# Autodesk Inventor assembly: Assembly_AIM
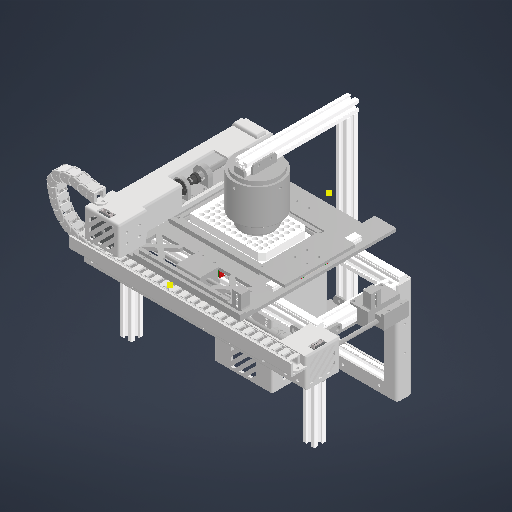
[picture p0: Inventor's stored thumbnail of the model, 512x512]
Saved by Autodesk Inventor 2026.2 (Build 302298000, 298)
## iProperties
Created: 2026-02-12
Part Number: Assembly_AIM
Document SubType Name: Assembly
Designer: Alvin
Author: Alvin
## Documents named in this file (54)
- C:\Users\Alvin\OneDrive\Documents\Inventor\NCKU_Automation_Incubator_Microscope\Assembly_AIM.iam
- C:\Users\Alvin\OneDrive\Documents\Inventor\NCKU_Automation_Incubator_Microscope\alpro base 200mm.ipt
- C:\Users\Alvin\OneDrive\Documents\Inventor\NCKU_Automation_Incubator_Microscope\alpro base 330mm.ipt
- C:\Users\Alvin\OneDrive\Documents\Inventor\NCKU_Automation_Incubator_Microscope\MGN12H_With_Rail x axis\MGN12H_With_Rail x axis.iam
- C:\Users\Alvin\OneDrive\Documents\Inventor\NCKU_Automation_Incubator_Microscope\stagex v7 new version\stagex v7 new version.iam
- C:\Users\Alvin\OneDrive\Documents\Inventor\NCKU_Automation_Incubator_Microscope\alpro base 120mm.ipt
- C:\Users\Alvin\OneDrive\Documents\Inventor\NCKU_Automation_Incubator_Microscope\bracketx.ipt
- C:\Users\Alvin\OneDrive\Documents\Inventor\NCKU_Automation_Incubator_Microscope\NEMA17 42-40\NEMA17 42-40\NEMA17 42-40.ipt
- C:\Users\Alvin\OneDrive\Documents\Inventor\NCKU_Automation_Incubator_Microscope\KFL08-KFL08-Part\KFL08-KFL08-Part.iam
- C:\Users\Alvin\OneDrive\Documents\Inventor\NCKU_Automation_Incubator_Microscope\MGN12H_With_Rail y axis\MGN12H_With_Rail y axis.iam
- C:\Users\Alvin\OneDrive\Documents\Inventor\NCKU_Automation_Incubator_Microscope\NEMA17_Coupler v1.ipt
- C:\Users\Alvin\OneDrive\Documents\Inventor\NCKU_Automation_Incubator_Microscope\8mm Threaded Rod 350mm.ipt
- C:\Users\Alvin\OneDrive\Documents\Inventor\NCKU_Automation_Incubator_Microscope\bracketx part2.ipt
- C:\Users\Alvin\OneDrive\Documents\Inventor\NCKU_Automation_Incubator_Microscope\anti-baclash nuts v1\anti-baclash nuts v1.iam
- C:\Users\Alvin\OneDrive\Documents\Inventor\NCKU_Automation_Incubator_Microscope\microswith.ipt
- C:\Users\Alvin\OneDrive\Documents\Inventor\NCKU_Automation_Incubator_Microscope\limitswitch_bracket_2 v1.ipt
- C:\Users\Alvin\OneDrive\Documents\Inventor\NCKU_Automation_Incubator_Microscope\plate assembly\plate assembly.iam
- C:\Users\Alvin\OneDrive\Documents\Inventor\NCKU_Automation_Incubator_Microscope\kfl_bracket_2 v1.ipt
- C:\Users\Alvin\OneDrive\Documents\Inventor\NCKU_Automation_Incubator_Microscope\brackety.ipt
- C:\Users\Alvin\OneDrive\Documents\Inventor\NCKU_Automation_Incubator_Microscope\8mm Threaded Rod 170mm.ipt
- C:\Users\Alvin\OneDrive\Documents\Inventor\NCKU_Automation_Incubator_Microscope\alpro base 290mm.ipt
- C:\Users\Alvin\OneDrive\Documents\Inventor\NCKU_Automation_Incubator_Microscope\z part new version.ipt
- C:\Users\Alvin\OneDrive\Documents\Inventor\NCKU_Automation_Incubator_Microscope\kfl_bracket v3.ipt
- C:\Users\Alvin\OneDrive\Documents\Inventor\NCKU_Automation_Incubator_Microscope\well plate\96 Well Plate, F-bottom, Standard v2.ipt
- C:\Users\Alvin\OneDrive\Documents\Inventor\NCKU_Automation_Incubator_Microscope\alpro base 400mm v4.ipt
- C:\Users\Alvin\OneDrive\Documents\Inventor\NCKU_Automation_Incubator_Microscope\8mm Threaded Rod 101.5mm.ipt
- C:\Users\Alvin\OneDrive\Documents\Inventor\NCKU_Automation_Incubator_Microscope\Metal rod 108mm (6mm).ipt
- C:\Users\Alvin\OneDrive\Documents\Inventor\NCKU_Automation_Incubator_Microscope\LMF8_fix.ipt
- C:\Users\Alvin\OneDrive\Documents\Inventor\NCKU_Automation_Incubator_Microscope\IModule_Mounting Part-2.ipt
- C:\Users\Alvin\OneDrive\Documents\Inventor\NCKU_Automation_Incubator_Microscope\IModule_Mounting Part-3.ipt
- C:\Users\Alvin\OneDrive\Documents\Inventor\NCKU_Automation_Incubator_Microscope\IModule_LED.ipt
- C:\Users\Alvin\OneDrive\Documents\Inventor\NCKU_Automation_Incubator_Microscope\IModule_Diffuser.ipt
- C:\Users\Alvin\OneDrive\Documents\Inventor\NCKU_Automation_Incubator_Microscope\IModule_CollectorLens.ipt
- C:\Users\Alvin\OneDrive\Documents\Inventor\NCKU_Automation_Incubator_Microscope\alpro base 220mm v4.ipt
- C:\Users\Alvin\OneDrive\Documents\Inventor\NCKU_Automation_Incubator_Microscope\IModule_Mounting Part-1.ipt
- C:\Users\Alvin\OneDrive\Documents\Inventor\NCKU_Automation_Incubator_Microscope\metal rod 180mm.ipt
- C:\Users\Alvin\OneDrive\Documents\Inventor\NCKU_Automation_Incubator_Microscope\10x Obj Lens Finite 160mm.ipt
- C:\Users\Alvin\OneDrive\Documents\Inventor\NCKU_Automation_Incubator_Microscope\z part 2 new version_1.ipt
- C:\Users\Alvin\OneDrive\Documents\Inventor\NCKU_Automation_Incubator_Microscope\Tube_ObjLens+RaspiCam.iam
- C:\Users\Alvin\OneDrive\Documents\Inventor\NCKU_Automation_Incubator_Microscope\raspberry-pi-global-shutter-camera-1.snapshot.4\Raspberry Pi Global Shutter Camera\Raspberry Pi Global Shutter Camera\Raspberry Pi.ipt
- C:\Users\Alvin\OneDrive\Documents\Inventor\NCKU_Automation_Incubator_Microscope\z_enclosure.ipt
- C:\Users\Alvin\OneDrive\Documents\Inventor\NCKU_Automation_Incubator_Microscope\xy_enclosure.ipt
- C:\Users\Alvin\OneDrive\Documents\Inventor\NCKU_Automation_Incubator_Microscope\x_enclosure.ipt
- C:\Users\Alvin\OneDrive\Documents\Inventor\NCKU_Automation_Incubator_Microscope\enclosure__bone_bottom.ipt
- C:\Users\Alvin\OneDrive\Documents\Inventor\NCKU_Automation_Incubator_Microscope\enclosure__bone_bottom_left.ipt
- C:\Users\Alvin\OneDrive\Documents\Inventor\NCKU_Automation_Incubator_Microscope\metal rod 80mm.ipt
- C:\Users\Alvin\OneDrive\Documents\Inventor\NCKU_Automation_Incubator_Microscope\chain_cable_male.ipt
- C:\Users\Alvin\OneDrive\Documents\Inventor\NCKU_Automation_Incubator_Microscope\chain_cable_mid.ipt
- C:\Users\Alvin\OneDrive\Documents\Inventor\NCKU_Automation_Incubator_Microscope\chain_cable_female.ipt
- C:\Users\Alvin\OneDrive\Documents\Inventor\NCKU_Automation_Incubator_Microscope\Assembly_AIM\AIP\FEA\feo31tnmo.fins
- C:\Users\Alvin\OneDrive\Documents\Inventor\NCKU_Automation_Incubator_Microscope\Assembly_AIM\AIP\FEA\feo31tnmo.fsat
- C:\Users\Alvin\OneDrive\Documents\Inventor\NCKU_Automation_Incubator_Microscope\Assembly_AIM\AIP\FEA\feo31tnmo.ftes
- C:\Users\Alvin\OneDrive\Documents\Inventor\NCKU_Automation_Incubator_Microscope\Assembly_AIM\AIP\FEA\feo31tnmo.fwiz
- C:\Users\Alvin\OneDrive\Documents\Inventor\NCKU_Automation_Incubator_Microscope\Assembly_AIM\AIP\FEA\feo31tq5c.fmsh
## Components (97 placed, 48 different names)
1. alpro base 330mm:1 — Flush:15, Flush:17, Mate:10, Mate:13, Flush:19, Flush:20, Mate:15, Flush:23, Flush:24, Mate:21, Flush:27, Mate:94, Flush:37, Mate:200, Flush:45, Flush:46, Mate:201, Flush:47, Flush:48
2. alpro base 330mm:2 — Flush:16, Flush:18, Mate:11, Mate:14, Flush:21, Flush:22, Mate:16, Flush:25, Flush:26, Mate:198, Flush:41, Flush:42, Mate:199, Flush:43, Flush:44
3. MGN12H_With_Rail x axis:1 [sub-assembly] — Flush:16, Flush:18, Mate:11, Mate:302, Mate:303, Mate:304
4. MGN12H_With_Rail x axis:2 [sub-assembly] — Flush:15, Flush:17, Mate:10, Mate:84
5. alpro base 120mm:1 — Mate:13, Flush:19, Flush:20, Mate:16, Flush:25, Flush:26, Mate:93
6. alpro base 120mm:2 — Mate:14, Flush:21, Flush:22, Mate:15, Flush:23, Flush:24, Mate:20, Mate:328, Mate:329
7. bracketx:1 — Mate:20, Mate:21, Flush:27, Mate:23, Mate:24, Mate:171, Mate:321, Mate:333
8. NEMA17 42-40:1 — Mate:23, Mate:24, Mate:38, Flush:29, Mate:171, Mate:335
9. NEMA17 42-40:2 — Mate:83, Flush:36, Mate:103, Mate:104, Mate:105, Mate:106, Mate:107
10. NEMA17 42-40:3 — Flush:30, Mate:56, Mate:284, Mate:285, Mate:286
11. MGN12H_With_Rail y axis:1 [sub-assembly] — Mate:58, Mate:59, Mate:290, Mate:291, Mate:292
12. MGN12H_With_Rail y axis:2 [sub-assembly] — Mate:57, Mate:60, Mate:61, Mate:287, Mate:288, Mate:289
13. NEMA17_Coupler v1:1 — Mate:83, Flush:36, Mate:118, Mate:119, Rotation:3, Mate:277
14. NEMA17_Coupler v1:2 — Flush:30, Mate:56, Cylindrical:5, Mate:75, Rotation:2
15. NEMA17_Coupler v1:3 — Mate:38, Flush:29, Cylindrical:2, Mate:39, Rotation:1
16. 8mm Threaded Rod 350mm:1 — Cylindrical:2, Mate:39, Rotation:1, Mate:45, Rotation/Translation:1, Mate:279
17. bracketx part2:1 — Mate:40, Mate:41, Mate:42, Mate:43, Mate:44, Rotation/Translation:1, Mate:84, Mate:195, Mate:196, Mate:296, Mate:297, Mate:298
18. anti-baclash nuts v1:1 [sub-assembly] — Mate:40, Mate:41, Mate:42, Mate:43, Mate:44, Mate:45
19. anti-baclash nuts v1:2 [sub-assembly] — Cylindrical:3, Mate:421, Mate:422, Mate:423
20. microswith:1 — Mate:299, Mate:301, Mate:316
21. microswith:2 — Mate:330, Mate:331, Mate:332
22. plate assembly:1 [sub-assembly] — Mate:57, Mate:58, Mate:59, Mate:60, Mate:61, Mate:233, Mate:234, Mate:235, Mate:418, Mate:419, Mate:420
23. kfl_bracket_2 v1:1 — Mate:71, Mate:72, Mate:73, Mate:74, Mate:305, Mate:306, Mate:309, Mate:416
24. KFL08-KFL08-Part:2 [sub-assembly] — Mate:71, Mate:72, Mate:73, Mate:74, Cylindrical:4
25. 8mm Threaded Rod 170mm:1 — Cylindrical:3, Cylindrical:4, Cylindrical:5, Mate:75, Rotation:2
26. kfl_bracket v3:1 — Mate:93, Mate:94, Flush:37, Mate:280, Mate:281, Mate:282
27. 96 Well Plate, F-bottom, Standard v2:1 — Mate:233, Mate:234, Mate:235
28. z part new version:1 — Mate:103, Mate:104, Mate:105, Mate:106, Mate:107, Mate:108, Flush:38, Mate:109, Mate:111, Mate:112, Mate:113, Mate:114, Mate:115, Mate:116, Mate:117, Mate:255, Mate:256, Flush:51, Flush:52, Mate:276, Mate:326, Mate:429
29. alpro base 400mm v4:1 — Mate:108, Flush:38, Mate:109, Mate:143, Flush:39, Flush:40
30. 8mm Threaded Rod 101.5mm:1 — Mate:117, Mate:118, Mate:119, Mate:140, Rotation:3
31. Metal rod 108mm (6mm):1 — Mate:111, Mate:112, Mate:113, Mate:142
32. Metal rod 108mm (6mm):2 — Mate:114, Mate:115, Mate:116, Mate:141
33. LMF8_fix:1 — Mate:142, Mate:262, Mate:267, Mate:268
34. LMF8_fix:2 — Mate:141, Mate:263, Mate:265, Mate:270
35. anti-baclash nuts v1:3 [sub-assembly] — Mate:140, Mate:264, Mate:266, Mate:269
36. alpro base 220mm v4:1 — Mate:143, Flush:39, Flush:40, Mate:163, Mate:244
37. IModule_CollectorLens:1 — Mate:149, Mate:153, Mate:154, Mate:155, Mate:156
38. IModule_Diffuser:1 — Mate:144, Mate:145
39. IModule_LED:1 — Mate:146, Mate:147, Mate:186, Mate:187
40. IModule_Mounting Part-1:1 — Mate:146, Mate:147, Mate:149, Mate:153, Mate:154, Mate:155, Mate:156, Mate:157, Mate:158, Mate:159, Mate:160, Mate:163, Mate:186, Mate:187, Mate:244
41. IModule_Mounting Part-2:1 — Mate:144, Mate:145, Mate:157, Mate:158, Mate:159, Mate:160, Mate:240, Mate:241, Mate:242, Mate:243, Mate:275, Mate:317
42. metal rod 180mm:1 — Mate:195, Mate:196, Mate:293, Mate:294, Mate:295
43. alpro base 200mm:1 — Mate:198, Flush:41, Flush:42, Flush:54, Mate:326
44. alpro base 200mm:2 — Mate:200, Flush:45, Flush:46
45. alpro base 200mm:3 — Mate:199, Flush:43, Flush:44, Mate:254, Flush:49, Flush:50, Mate:324
46. alpro base 200mm:4 — Mate:201, Flush:47, Flush:48
47. Raspberry Pi:1 — Mate:259, Mate:260, Mate:272, Mate:273, Mate:274
48. IModule_Mounting Part-3:1 — Mate:240, Mate:241, Mate:242, Mate:243
49. alpro base 290mm:1 — Mate:254, Flush:49, Flush:50, Mate:255, Mate:256, Mate:323, Flush:55, Mate:325
50. 10x Obj Lens Finite 160mm:1 — Mate:257, Mate:258, Mate:275, Mate:317
51. Tube_ObjLens+RaspiCam:1 [sub-assembly] — Mate:257, Mate:258, Mate:259, Mate:260, Mate:271
52. z part 2 new version_1:1 — Mate:262, Mate:263, Mate:264, Mate:265, Mate:266, Mate:267, Mate:268, Mate:269, Mate:270, Mate:271, Mate:272, Mate:273, Mate:274, Mate:277
53. z_enclosure:1 — Flush:51, Flush:52, Mate:276
54. KFL08-KFL08-Part:3 [sub-assembly] — Mate:279, Mate:280, Mate:281, Mate:282
55. stagex v7 new version:1 [sub-assembly] — Mate:284, Mate:285, Mate:286, Mate:287, Mate:288, Mate:289, Mate:290, Mate:291, Mate:292, Mate:293, Mate:294, Mate:295, Mate:296, Mate:297, Mate:298, Mate:299, Mate:301, Mate:302, Mate:303, Mate:304, Mate:305, Mate:306, Mate:309, Mate:316, Mate:416, Mate:424, Mate:425, Mate:426
56. x_enclosure:1 — Mate:321, Mate:370, Mate:371, Mate:415
57. enclosure__bone_bottom:1 — Flush:54, Mate:323
58. enclosure__bone_bottom_left:1 — Flush:55, Mate:324, Mate:325, Mate:429
59. limitswitch_bracket_2 v1:1 — Mate:328, Mate:329, Mate:330, Mate:331, Mate:332, Flush:56
60. metal rod 80mm:1 — Mate:333, Mate:335, Flush:56, Mate:415
61. chain_cable_female:1 — Mate:409, Flush:94, Mate:427, Mate:428
62. chain_cable_male:1 — Mate:370, Mate:371, Mate:372, Flush:62
63. chain_cable_mid:13 — Mate:372, Flush:62, Mate:373, Flush:63
64. chain_cable_mid:14 — Mate:373, Flush:63, Mate:375, Flush:65
65. chain_cable_mid:15 — Mate:375, Flush:65
66. chain_cable_mid:16 — Mate:379, Flush:69
67. chain_cable_mid:17 — Mate:379, Flush:69
68. chain_cable_mid:18
69. chain_cable_mid:19
70. chain_cable_mid:20 — Mate:387, Flush:77
71. chain_cable_mid:21 — Mate:387, Flush:77
72. chain_cable_mid:22
73. chain_cable_mid:23
74. chain_cable_mid:24
75. chain_cable_mid:25
76. chain_cable_mid:26
77. chain_cable_mid:27
78. chain_cable_mid:28 — Mate:403, Flush:93
79. chain_cable_mid:29 — Mate:403, Flush:93
80. chain_cable_mid:30
81. chain_cable_mid:31
82. chain_cable_mid:32
83. chain_cable_mid:33
84. chain_cable_mid:34
85. chain_cable_mid:35
86. chain_cable_mid:36
87. chain_cable_mid:37
88. chain_cable_mid:38
89. chain_cable_mid:39
90. chain_cable_mid:40
91. chain_cable_mid:41 — Mate:413, Flush:98
92. chain_cable_mid:43 — Mate:409, Flush:94, Mate:412, Flush:97
93. chain_cable_mid:44 — Mate:410, Flush:95, Mate:411, Flush:96
94. chain_cable_mid:45 — Mate:410, Flush:95, Mate:412, Flush:97
95. chain_cable_mid:46 — Mate:411, Flush:96, Mate:413, Flush:98
96. brackety:1 — Mate:418, Mate:419, Mate:420, Mate:421, Mate:422, Mate:423
97. xy_enclosure:1 — Mate:424, Mate:425, Mate:426, Mate:427, Mate:428
## Relationships (275: Mate 198, Flush 69, CylindricalJoint 4, RelateRotation 3, RelateRotateTranslate 1)
- Flush:15: alpro base 330mm:1 ↔ MGN12H_With_Rail x axis:2
- Flush:16: alpro base 330mm:2 ↔ MGN12H_With_Rail x axis:1
- Flush:17 (4 mm): alpro base 330mm:1 ↔ MGN12H_With_Rail x axis:2
- Flush:18 (4 mm): alpro base 330mm:2 ↔ MGN12H_With_Rail x axis:1
- Mate:10: alpro base 330mm:1 ↔ MGN12H_With_Rail x axis:2
- Mate:11: alpro base 330mm:2 ↔ MGN12H_With_Rail x axis:1
- Mate:13: alpro base 330mm:1 ↔ alpro base 120mm:1
- Flush:19: alpro base 330mm:1 ↔ alpro base 120mm:1
- Flush:20: alpro base 330mm:1 ↔ alpro base 120mm:1
- Mate:14: alpro base 330mm:2 ↔ alpro base 120mm:2
- Flush:21: alpro base 330mm:2 ↔ alpro base 120mm:2
- Flush:22: alpro base 330mm:2 ↔ alpro base 120mm:2
- Mate:15: alpro base 330mm:1 ↔ alpro base 120mm:2
- Flush:23: alpro base 330mm:1 ↔ alpro base 120mm:2
- Flush:24: alpro base 330mm:1 ↔ alpro base 120mm:2
- Mate:16: alpro base 330mm:2 ↔ alpro base 120mm:1
- Flush:25: alpro base 330mm:2 ↔ alpro base 120mm:1
- Flush:26: alpro base 330mm:2 ↔ alpro base 120mm:1
- Mate:20: alpro base 120mm:2 ↔ bracketx:1
- Mate:21: alpro base 330mm:1 ↔ bracketx:1
- Flush:27 (3 mm): alpro base 330mm:1 ↔ bracketx:1
- Mate:23: bracketx:1 ↔ NEMA17 42-40:1
- Mate:24: bracketx:1 ↔ NEMA17 42-40:1
- Mate:38: NEMA17 42-40:1 ↔ NEMA17_Coupler v1:3
- Flush:29: NEMA17 42-40:1 ↔ NEMA17_Coupler v1:3
- Cylindrical:2: NEMA17_Coupler v1:3 ↔ 8mm Threaded Rod 350mm:1
- Mate:39: NEMA17_Coupler v1:3 ↔ 8mm Threaded Rod 350mm:1
- Rotation:1 [RelateRotation] (0.977 ul): NEMA17_Coupler v1:3 ↔ 8mm Threaded Rod 350mm:1
- Mate:40: bracketx part2:1 ↔ anti-baclash nuts v1:1
- Mate:41: bracketx part2:1 ↔ anti-baclash nuts v1:1
- Mate:42: bracketx part2:1 ↔ anti-baclash nuts v1:1
- Mate:43: bracketx part2:1 ↔ anti-baclash nuts v1:1
- Mate:44: bracketx part2:1 ↔ anti-baclash nuts v1:1
- Mate:45: 8mm Threaded Rod 350mm:1 ↔ anti-baclash nuts v1:1
- Rotation/Translation:1 [RelateRotateTranslate] (8 mm): 8mm Threaded Rod 350mm:1 ↔ bracketx part2:1
- Flush:30: NEMA17 42-40:3 ↔ NEMA17_Coupler v1:2
- Mate:56: NEMA17 42-40:3 ↔ NEMA17_Coupler v1:2
- Mate:57: MGN12H_With_Rail y axis:2 ↔ plate assembly:1
- Mate:58: MGN12H_With_Rail y axis:1 ↔ plate assembly:1
- Mate:59: MGN12H_With_Rail y axis:1 ↔ plate assembly:1
- Mate:60: MGN12H_With_Rail y axis:2 ↔ plate assembly:1
- Mate:61: MGN12H_With_Rail y axis:2 ↔ plate assembly:1
- Mate:71: kfl_bracket_2 v1:1 ↔ KFL08-KFL08-Part:2
- Mate:72: kfl_bracket_2 v1:1 ↔ KFL08-KFL08-Part:2
- Mate:73: kfl_bracket_2 v1:1 ↔ KFL08-KFL08-Part:2
- Mate:74: kfl_bracket_2 v1:1 ↔ KFL08-KFL08-Part:2
- Cylindrical:3: anti-baclash nuts v1:2 ↔ 8mm Threaded Rod 170mm:1
- Cylindrical:4: KFL08-KFL08-Part:2 ↔ 8mm Threaded Rod 170mm:1
- Cylindrical:5: NEMA17_Coupler v1:2 ↔ 8mm Threaded Rod 170mm:1
- Mate:75: NEMA17_Coupler v1:2 ↔ 8mm Threaded Rod 170mm:1
- Rotation:2 [RelateRotation] (2.543 ul): NEMA17_Coupler v1:2 ↔ 8mm Threaded Rod 170mm:1
- Mate:83: NEMA17 42-40:2 ↔ NEMA17_Coupler v1:1
- Flush:36: NEMA17 42-40:2 ↔ NEMA17_Coupler v1:1
- Mate:84: MGN12H_With_Rail x axis:2 ↔ bracketx part2:1
- Mate:93: alpro base 120mm:1 ↔ kfl_bracket v3:1
- Mate:94: alpro base 330mm:1 ↔ kfl_bracket v3:1
- Flush:37 (3 mm): alpro base 330mm:1 ↔ kfl_bracket v3:1
- Mate:103: NEMA17 42-40:2 ↔ z part new version:1
- Mate:104: NEMA17 42-40:2 ↔ z part new version:1
- Mate:105: NEMA17 42-40:2 ↔ z part new version:1
- Mate:106: NEMA17 42-40:2 ↔ z part new version:1
- Mate:107: NEMA17 42-40:2 ↔ z part new version:1
- Mate:108: z part new version:1 ↔ alpro base 400mm v4:1
- Flush:38: z part new version:1 ↔ alpro base 400mm v4:1
- Mate:109: z part new version:1 ↔ alpro base 400mm v4:1
- Mate:111: z part new version:1 ↔ Metal rod 108mm (6mm):1
- Mate:112: z part new version:1 ↔ Metal rod 108mm (6mm):1
- Mate:113: z part new version:1 ↔ Metal rod 108mm (6mm):1
- Mate:114: z part new version:1 ↔ Metal rod 108mm (6mm):2
- Mate:115: z part new version:1 ↔ Metal rod 108mm (6mm):2
- Mate:116: z part new version:1 ↔ Metal rod 108mm (6mm):2
- Mate:117: z part new version:1 ↔ 8mm Threaded Rod 101.5mm:1
- Mate:118: NEMA17_Coupler v1:1 ↔ 8mm Threaded Rod 101.5mm:1
- Mate:119: NEMA17_Coupler v1:1 ↔ 8mm Threaded Rod 101.5mm:1
- Mate:140: 8mm Threaded Rod 101.5mm:1 ↔ anti-baclash nuts v1:3
- Mate:141: Metal rod 108mm (6mm):2 ↔ LMF8_fix:2
- Mate:142: Metal rod 108mm (6mm):1 ↔ LMF8_fix:1
- Rotation:3 [RelateRotation] (0.393 ul): NEMA17_Coupler v1:1 ↔ 8mm Threaded Rod 101.5mm:1
- Mate:143: alpro base 400mm v4:1 ↔ alpro base 220mm v4:1
- Flush:39: alpro base 400mm v4:1 ↔ alpro base 220mm v4:1
- Flush:40: alpro base 400mm v4:1 ↔ alpro base 220mm v4:1
- Mate:144: IModule_Diffuser:1 ↔ IModule_Mounting Part-2:1
- Mate:145: IModule_Diffuser:1 ↔ IModule_Mounting Part-2:1
- Mate:146: IModule_LED:1 ↔ IModule_Mounting Part-1:1
- Mate:147: IModule_LED:1 ↔ IModule_Mounting Part-1:1
- Mate:149: IModule_CollectorLens:1 ↔ IModule_Mounting Part-1:1
- Mate:153: IModule_CollectorLens:1 ↔ IModule_Mounting Part-1:1
- Mate:154: IModule_CollectorLens:1 ↔ IModule_Mounting Part-1:1
- Mate:155: IModule_CollectorLens:1 ↔ IModule_Mounting Part-1:1
- Mate:156: IModule_CollectorLens:1 ↔ IModule_Mounting Part-1:1
- Mate:157: IModule_Mounting Part-1:1 ↔ IModule_Mounting Part-2:1
- Mate:158: IModule_Mounting Part-1:1 ↔ IModule_Mounting Part-2:1
- Mate:159: IModule_Mounting Part-1:1 ↔ IModule_Mounting Part-2:1
- Mate:160: IModule_Mounting Part-1:1 ↔ IModule_Mounting Part-2:1
- Mate:163: alpro base 220mm v4:1 ↔ IModule_Mounting Part-1:1
- Mate:171: bracketx:1 ↔ NEMA17 42-40:1
- Mate:186: IModule_LED:1 ↔ IModule_Mounting Part-1:1
- Mate:187: IModule_LED:1 ↔ IModule_Mounting Part-1:1
- Mate:195: bracketx part2:1 ↔ metal rod 180mm:1
- Mate:196: bracketx part2:1 ↔ metal rod 180mm:1
- Mate:198: alpro base 330mm:2 ↔ alpro base 200mm:1
- Flush:41: alpro base 330mm:2 ↔ alpro base 200mm:1
- Flush:42: alpro base 330mm:2 ↔ alpro base 200mm:1
- Mate:199: alpro base 330mm:2 ↔ alpro base 200mm:3
- Flush:43: alpro base 330mm:2 ↔ alpro base 200mm:3
- Flush:44: alpro base 330mm:2 ↔ alpro base 200mm:3
- Mate:200: alpro base 330mm:1 ↔ alpro base 200mm:2
- Flush:45: alpro base 330mm:1 ↔ alpro base 200mm:2
- Flush:46: alpro base 330mm:1 ↔ alpro base 200mm:2
- Mate:201: alpro base 330mm:1 ↔ alpro base 200mm:4
- Flush:47: alpro base 330mm:1 ↔ alpro base 200mm:4
- Flush:48: alpro base 330mm:1 ↔ alpro base 200mm:4
- Mate:233: plate assembly:1 ↔ 96 Well Plate, F-bottom, Standard v2:1
- Mate:234: plate assembly:1 ↔ 96 Well Plate, F-bottom, Standard v2:1
- Mate:235: plate assembly:1 ↔ 96 Well Plate, F-bottom, Standard v2:1
- Mate:240: IModule_Mounting Part-2:1 ↔ IModule_Mounting Part-3:1
- Mate:241: IModule_Mounting Part-2:1 ↔ IModule_Mounting Part-3:1
- Mate:242: IModule_Mounting Part-2:1 ↔ IModule_Mounting Part-3:1
- Mate:243: IModule_Mounting Part-2:1 ↔ IModule_Mounting Part-3:1
- Mate:244: alpro base 220mm v4:1 ↔ IModule_Mounting Part-1:1
- Mate:254: alpro base 200mm:3 ↔ alpro base 290mm:1
- Flush:49: alpro base 200mm:3 ↔ alpro base 290mm:1
- Flush:50: alpro base 200mm:3 ↔ alpro base 290mm:1
- Mate:255: z part new version:1 ↔ alpro base 290mm:1
- Mate:256: z part new version:1 ↔ alpro base 290mm:1
- Mate:257: 10x Obj Lens Finite 160mm:1 ↔ Tube_ObjLens+RaspiCam:1
- Mate:258: 10x Obj Lens Finite 160mm:1 ↔ Tube_ObjLens+RaspiCam:1
- Mate:259: Raspberry Pi:1 ↔ Tube_ObjLens+RaspiCam:1
- Mate:260: Raspberry Pi:1 ↔ Tube_ObjLens+RaspiCam:1
- Mate:262: LMF8_fix:1 ↔ z part 2 new version_1:1
- Mate:263: LMF8_fix:2 ↔ z part 2 new version_1:1
- Mate:264: anti-baclash nuts v1:3 ↔ z part 2 new version_1:1
- Mate:265: LMF8_fix:2 ↔ z part 2 new version_1:1
- Mate:266: anti-baclash nuts v1:3 ↔ z part 2 new version_1:1
- Mate:267: LMF8_fix:1 ↔ z part 2 new version_1:1
- Mate:268: LMF8_fix:1 ↔ z part 2 new version_1:1
- Mate:269: anti-baclash nuts v1:3 ↔ z part 2 new version_1:1
- Mate:270: LMF8_fix:2 ↔ z part 2 new version_1:1
- Mate:271: Tube_ObjLens+RaspiCam:1 ↔ z part 2 new version_1:1
- Mate:272: Raspberry Pi:1 ↔ z part 2 new version_1:1
- Mate:273: Raspberry Pi:1 ↔ z part 2 new version_1:1
- Mate:274: Raspberry Pi:1 ↔ z part 2 new version_1:1
- Mate:275: IModule_Mounting Part-2:1 ↔ 10x Obj Lens Finite 160mm:1
- Flush:51: z part new version:1 ↔ z_enclosure:1
- Flush:52: z part new version:1 ↔ z_enclosure:1
- Mate:276: z part new version:1 ↔ z_enclosure:1
- Mate:277: NEMA17_Coupler v1:1 ↔ z part 2 new version_1:1
- Mate:279: 8mm Threaded Rod 350mm:1 ↔ KFL08-KFL08-Part:3
- Mate:280: kfl_bracket v3:1 ↔ KFL08-KFL08-Part:3
- Mate:281: kfl_bracket v3:1 ↔ KFL08-KFL08-Part:3
- Mate:282: kfl_bracket v3:1 ↔ KFL08-KFL08-Part:3
- Mate:284: NEMA17 42-40:3 ↔ stagex v7 new version:1
- Mate:285: NEMA17 42-40:3 ↔ stagex v7 new version:1
- Mate:286: NEMA17 42-40:3 ↔ stagex v7 new version:1
- Mate:287: MGN12H_With_Rail y axis:2 ↔ stagex v7 new version:1
- Mate:288: MGN12H_With_Rail y axis:2 ↔ stagex v7 new version:1
- Mate:289: MGN12H_With_Rail y axis:2 ↔ stagex v7 new version:1
- Mate:290: MGN12H_With_Rail y axis:1 ↔ stagex v7 new version:1
- Mate:291: MGN12H_With_Rail y axis:1 ↔ stagex v7 new version:1
- Mate:292: MGN12H_With_Rail y axis:1 ↔ stagex v7 new version:1
- Mate:293: metal rod 180mm:1 ↔ stagex v7 new version:1
- Mate:294: metal rod 180mm:1 ↔ stagex v7 new version:1
- Mate:295: metal rod 180mm:1 ↔ stagex v7 new version:1
- Mate:296: bracketx part2:1 ↔ stagex v7 new version:1
- Mate:297: bracketx part2:1 ↔ stagex v7 new version:1
- Mate:298: bracketx part2:1 ↔ stagex v7 new version:1
- Mate:299: microswith:1 ↔ stagex v7 new version:1
- Mate:301: microswith:1 ↔ stagex v7 new version:1
- Mate:302: MGN12H_With_Rail x axis:1 ↔ stagex v7 new version:1
- Mate:303: MGN12H_With_Rail x axis:1 ↔ stagex v7 new version:1
- Mate:304: MGN12H_With_Rail x axis:1 ↔ stagex v7 new version:1
- Mate:305: kfl_bracket_2 v1:1 ↔ stagex v7 new version:1
- Mate:306: kfl_bracket_2 v1:1 ↔ stagex v7 new version:1
- Mate:309: kfl_bracket_2 v1:1 ↔ stagex v7 new version:1
- Mate:316: microswith:1 ↔ stagex v7 new version:1
- Mate:317: IModule_Mounting Part-2:1 ↔ 10x Obj Lens Finite 160mm:1
- Mate:321: bracketx:1 ↔ x_enclosure:1
- Flush:54: alpro base 200mm:1 ↔ enclosure__bone_bottom:1
- Mate:323: alpro base 290mm:1 ↔ enclosure__bone_bottom:1
- Flush:55: alpro base 290mm:1 ↔ enclosure__bone_bottom_left:1
- Mate:324: alpro base 200mm:3 ↔ enclosure__bone_bottom_left:1
- Mate:325: alpro base 290mm:1 ↔ enclosure__bone_bottom_left:1
- Mate:326 (100 mm): z part new version:1 ↔ alpro base 200mm:1
- Mate:328: alpro base 120mm:2 ↔ limitswitch_bracket_2 v1:1
- Mate:329: alpro base 120mm:2 ↔ limitswitch_bracket_2 v1:1
- Mate:330: microswith:2 ↔ limitswitch_bracket_2 v1:1
- Mate:331: microswith:2 ↔ limitswitch_bracket_2 v1:1
- Mate:332: microswith:2 ↔ limitswitch_bracket_2 v1:1
- Mate:333: bracketx:1 ↔ metal rod 80mm:1
- Mate:335: NEMA17 42-40:1 ↔ metal rod 80mm:1
- Flush:56: limitswitch_bracket_2 v1:1 ↔ metal rod 80mm:1
- Mate:370: x_enclosure:1 ↔ chain_cable_male:1
- Mate:371: x_enclosure:1 ↔ chain_cable_male:1
- Mate:372: chain_cable_male:1 ↔ chain_cable_mid:13
- Flush:62: chain_cable_male:1 ↔ chain_cable_mid:13
- Mate:373: chain_cable_mid:13 ↔ chain_cable_mid:14
- Flush:63: chain_cable_mid:13 ↔ chain_cable_mid:14
- [Mate]: chain_cable_mid:15 ↔ chain_cable_mid:16
- [Flush]: chain_cable_mid:15 ↔ chain_cable_mid:16
- Mate:375: chain_cable_mid:14 ↔ chain_cable_mid:15
- Flush:65: chain_cable_mid:14 ↔ chain_cable_mid:15
- [Mate]: chain_cable_mid:17 ↔ chain_cable_mid:18
- [Flush]: chain_cable_mid:17 ↔ chain_cable_mid:18
- [Mate]: chain_cable_mid:19 ↔ chain_cable_mid:20
- [Flush]: chain_cable_mid:19 ↔ chain_cable_mid:20
- [Mate]: chain_cable_mid:18 ↔ chain_cable_mid:19
- [Flush]: chain_cable_mid:18 ↔ chain_cable_mid:19
- Mate:379: chain_cable_mid:16 ↔ chain_cable_mid:17
- Flush:69: chain_cable_mid:16 ↔ chain_cable_mid:17
- [Mate]: chain_cable_mid:21 ↔ chain_cable_mid:22
- [Flush]: chain_cable_mid:21 ↔ chain_cable_mid:22
- [Mate]: chain_cable_mid:23 ↔ chain_cable_mid:24
- [Flush]: chain_cable_mid:23 ↔ chain_cable_mid:24
- [Mate]: chain_cable_mid:22 ↔ chain_cable_mid:23
- [Flush]: chain_cable_mid:22 ↔ chain_cable_mid:23
- [Mate]: chain_cable_mid:25 ↔ chain_cable_mid:26
- [Flush]: chain_cable_mid:25 ↔ chain_cable_mid:26
- [Mate]: chain_cable_mid:27 ↔ chain_cable_mid:28
- [Flush]: chain_cable_mid:27 ↔ chain_cable_mid:28
- [Mate]: chain_cable_mid:26 ↔ chain_cable_mid:27
- [Flush]: chain_cable_mid:26 ↔ chain_cable_mid:27
- [Mate]: chain_cable_mid:24 ↔ chain_cable_mid:25
- [Flush]: chain_cable_mid:24 ↔ chain_cable_mid:25
- Mate:387: chain_cable_mid:20 ↔ chain_cable_mid:21
- Flush:77: chain_cable_mid:20 ↔ chain_cable_mid:21
- [Mate]: chain_cable_mid:29 ↔ chain_cable_mid:30
- [Flush]: chain_cable_mid:29 ↔ chain_cable_mid:30
- [Mate]: chain_cable_mid:31 ↔ chain_cable_mid:32
- [Flush]: chain_cable_mid:31 ↔ chain_cable_mid:32
- [Mate]: chain_cable_mid:30 ↔ chain_cable_mid:31
- [Flush]: chain_cable_mid:30 ↔ chain_cable_mid:31
- [Mate]: chain_cable_mid:33 ↔ chain_cable_mid:34
- [Flush]: chain_cable_mid:33 ↔ chain_cable_mid:34
- [Mate]: chain_cable_mid:35 ↔ chain_cable_mid:36
- [Flush]: chain_cable_mid:35 ↔ chain_cable_mid:36
- [Mate]: chain_cable_mid:34 ↔ chain_cable_mid:35
- [Flush]: chain_cable_mid:34 ↔ chain_cable_mid:35
- [Mate]: chain_cable_mid:32 ↔ chain_cable_mid:33
- [Flush]: chain_cable_mid:32 ↔ chain_cable_mid:33
- [Mate]: chain_cable_mid:37 ↔ chain_cable_mid:38
- [Flush]: chain_cable_mid:37 ↔ chain_cable_mid:38
- [Mate]: chain_cable_mid:39 ↔ chain_cable_mid:40
- [Flush]: chain_cable_mid:39 ↔ chain_cable_mid:40
- [Mate]: chain_cable_mid:38 ↔ chain_cable_mid:39
- [Flush]: chain_cable_mid:38 ↔ chain_cable_mid:39
- [Mate]: chain_cable_mid:40 ↔ chain_cable_mid:41
- [Flush]: chain_cable_mid:40 ↔ chain_cable_mid:41
- [Mate]: chain_cable_mid:36 ↔ chain_cable_mid:37
- [Flush]: chain_cable_mid:36 ↔ chain_cable_mid:37
- Mate:403: chain_cable_mid:28 ↔ chain_cable_mid:29
- Flush:93: chain_cable_mid:28 ↔ chain_cable_mid:29
- Mate:409: chain_cable_female:1 ↔ chain_cable_mid:43
- Flush:94: chain_cable_female:1 ↔ chain_cable_mid:43
- Mate:410: chain_cable_mid:44 ↔ chain_cable_mid:45
- Flush:95: chain_cable_mid:44 ↔ chain_cable_mid:45
- Mate:411: chain_cable_mid:44 ↔ chain_cable_mid:46
- Flush:96: chain_cable_mid:44 ↔ chain_cable_mid:46
- Mate:412: chain_cable_mid:43 ↔ chain_cable_mid:45
- Flush:97: chain_cable_mid:43 ↔ chain_cable_mid:45
- Mate:413: chain_cable_mid:41 ↔ chain_cable_mid:46
- Flush:98: chain_cable_mid:41 ↔ chain_cable_mid:46
- Mate:415: x_enclosure:1 ↔ metal rod 80mm:1
- Mate:416: kfl_bracket_2 v1:1 ↔ stagex v7 new version:1
- Mate:418: plate assembly:1 ↔ brackety:1
- Mate:419: plate assembly:1 ↔ brackety:1
- Mate:420: plate assembly:1 ↔ brackety:1
- Mate:421: anti-baclash nuts v1:2 ↔ brackety:1
- Mate:422: anti-baclash nuts v1:2 ↔ brackety:1
- Mate:423: anti-baclash nuts v1:2 ↔ brackety:1
- Mate:424: stagex v7 new version:1 ↔ xy_enclosure:1
- Mate:425: stagex v7 new version:1 ↔ xy_enclosure:1
- Mate:426: stagex v7 new version:1 ↔ xy_enclosure:1
- Mate:427: chain_cable_female:1 ↔ xy_enclosure:1
- Mate:428: chain_cable_female:1 ↔ xy_enclosure:1
- Mate:429: z part new version:1 ↔ enclosure__bone_bottom_left:1
## Named parameters: d668_d666 = 0 mm, d669_d667 = 0 mm, d672_d666 = 0 mm, d673_d667 = 0 mm, d674_d668_d666 = 0 mm, d675_d669_d667 = 0 mm, d676_d670 = 0 mm, d677_d671 = 0 mm, d680_d666 = 0 mm, d681_d667 = 0 mm, d682_d668_d666 = 0 mm, d683_d669_d667 = 0 mm, d684_d670 = 0 mm, d685_d671 = 0 mm, d686_d672_d666 = 0 mm, d687_d673_d667 = 0 mm, d688_d674_d668_d666 = 0 mm, d689_d675_d669_d667 = 0 mm, d690_d676_d670 = 0 mm, d691_d677_d671 = 0 mm, d692_d678 = 0 mm, d693_d679 = 0 mm, d696_d666 = 0 mm, d697_d667 = 0 mm, d698_d668_d666 = 0 mm, d699_d669_d667 = 0 mm, d700_d670 = 0 mm, d701_d671 = 0 mm, d702_d672_d666 = 0 mm, d703_d673_d667 = 0 mm, d704_d674_d668_d666 = 0 mm, d705_d675_d669_d667 = 0 mm, d706_d676_d670 = 0 mm, d707_d677_d671 = 0 mm, d708_d678 = 0 mm, d709_d679 = 0 mm, d710_d680_d666 = 0 mm, d711_d681_d667 = 0 mm, d712_d682_d668_d666 = 0 mm, d713_d683_d669_d667 = 0 mm, d714_d684_d670 = 0 mm, d715_d685_d671 = 0 mm, d722_d692_d678 = 0 mm, d723_d693_d679 = 0 mm, d724_d694 = 0 mm, d725_d695 = 0 mm, sa_0 = 981
note: some values were not read from the file. Shown as the stored number, unit unknown: "sa_0".
